# Autodesk Inventor assembly: Assembly1
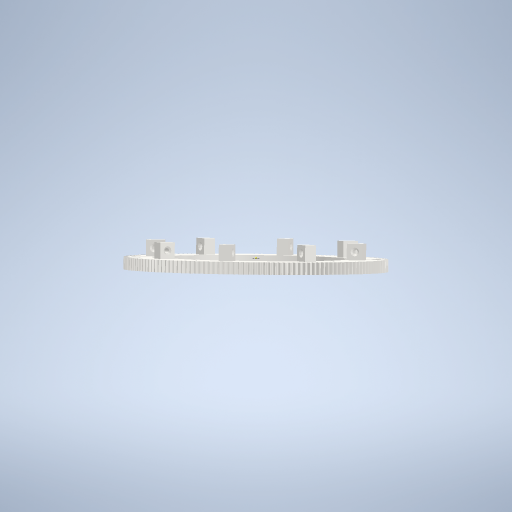
[picture p0: Inventor's stored thumbnail of the model, 512x512]
Saved by Autodesk Inventor 2023 (Build 270158000, 158)
## iProperties
Created: 2023-04-05
Part Number: Assembly1
Document SubType Name: Assembly
Designer: czapa
Author: czapa
## Documents named in this file (2)
- C:\Users\czapa\OneDrive\Documents\GitHub\S.P.I.C.E\3D Models\Version1\stls\Assembly1.iam
- C:\Users\czapa\OneDrive\Documents\GitHub\S.P.I.C.E\3D Models\Version1\BearingGearMk2.ipt
## Components (2 placed, 1 different names)
1. Spur Gear2:1 — Flush:1, Mate:1
2. Spur Gear2:2 — Flush:1, Mate:1
## Relationships (2: Flush 1, Mate 1)
- Flush:1: Spur Gear2:1 ↔ Spur Gear2:2
- Mate:1: Spur Gear2:1 ↔ Spur Gear2:2
